# Autodesk Inventor assembly: AM14U3 Wide Frame Wheel mount
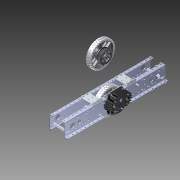
[picture p0: Inventor's stored thumbnail of the model, 180x180]
Saved by Autodesk Inventor 2014 (Build 180170000, 170)
## iProperties
Created: 2016-01-19
Part Number: AM14U3 Wide Frame Wheel mount
Document SubType Name: Assembly
Designer: choices
Author: choices
## Documents named in this file (12)
- F:\Robotics who knows idk\2016 Robot CAD Files\AndyMark Chassis things\AM14U3 Wide Frame Wheel mount.iam
- F:\Robotics who knows idk\2016 Robot CAD Files\AndyMark Chassis things\Churro 3375.ipt
- F:\Robotics who knows idk\2016 Robot CAD Files\AndyMark Chassis things\FHTS 0.25-20-0.75_FHTS 0.25-20-G-0.75-C.ipt
- F:\Robotics who knows idk\2016 Robot CAD Files\AndyMark Chassis things\10-32x0500_shcs_HX-SHCS 0.19-32x1.375x1-C.ipt
- F:\Robotics who knows idk\2016 Robot CAD Files\AndyMark Chassis things\10-32 Nylock Nut.ipt
- F:\Robotics who knows idk\2016 Robot CAD Files\AndyMark Chassis things\AM14U3 Outside Sheet Wide.ipt
- F:\Robotics who knows idk\2016 Robot CAD Files\AndyMark Chassis things\AM14U3 Inside Sheet Wide.ipt
- F:\Robotics who knows idk\2016 Robot CAD Files\AndyMark Chassis things\am-2954 AM14U2 2x3 Hole Bracket.ipt
- F:\Robotics who knows idk\2016 Robot CAD Files\AndyMark Chassis things\6 HiGrip with hub and double pulley.iam
- F:\Robotics who knows idk\2016 Robot CAD Files\AndyMark Chassis things\FR8ZZ Hex Bearing.ipt
- F:\Robotics who knows idk\2016 Robot CAD Files\AndyMark Chassis things\am-2598_107 2016 KOP Toughbox Mini.iam
- F:\Robotics who knows idk\2016 Robot CAD Files\AndyMark Chassis things\6 HiGrip with bearings, pulleys and spacers.iam
## Components (47 placed, 47 different names)
1. Churro 3375_80
2. Churro 3375_81
3. Churro 3375_82
4. Churro 3375_83
5. FHTS 0.25-20-0.75_FHTS 0.25-20-G-0.75-C_85
6. FHTS 0.25-20-0.75_FHTS 0.25-20-G-0.75-C_86
7. FHTS 0.25-20-0.75_FHTS 0.25-20-G-0.75-C_87
8. FHTS 0.25-20-0.75_FHTS 0.25-20-G-0.75-C_88
9. FHTS 0.25-20-0.75_FHTS 0.25-20-G-0.75-C_89
10. FHTS 0.25-20-0.75_FHTS 0.25-20-G-0.75-C_90
11. FHTS 0.25-20-0.75_FHTS 0.25-20-G-0.75-C_91
12. FHTS 0.25-20-0.75_FHTS 0.25-20-G-0.75-C_92
13. FHTS 0.25-20-0.75_FHTS 0.25-20-G-0.75-C_93
14. 10-32x0500_shcs_HX-SHCS 0.19-32x1.375x1-C_95
15. 10-32x0500_shcs_HX-SHCS 0.19-32x1.375x1-C_96
16. 10-32x0500_shcs_HX-SHCS 0.19-32x1.375x1-C_97
17. 10-32x0500_shcs_HX-SHCS 0.19-32x1.375x1-C_98
18. 10-32x0500_shcs_HX-SHCS 0.19-32x1.375x1-C_99
19. 10-32x0500_shcs_HX-SHCS 0.19-32x1.375x1-C_100
20. 10-32x0500_shcs_HX-SHCS 0.19-32x1.375x1-C_101
21. 10-32x0500_shcs_HX-SHCS 0.19-32x1.375x1-C_102
22. 10-32x0500_shcs_HX-SHCS 0.19-32x1.375x1-C_103
23. 10-32x0500_shcs_HX-SHCS 0.19-32x1.375x1-C_104
24. 10-32x0500_shcs_HX-SHCS 0.19-32x1.375x1-C_105
25. 10-32x0500_shcs_HX-SHCS 0.19-32x1.375x1-C_106
26. 10-32x0500_shcs_HX-SHCS 0.19-32x1.375x1-C_107
27. 10-32 Nylock Nut_113
28. 10-32 Nylock Nut_114
29. 10-32 Nylock Nut_115
30. 10-32 Nylock Nut_116
31. 10-32 Nylock Nut_117
32. 10-32 Nylock Nut_118
33. 10-32 Nylock Nut_119
34. 10-32 Nylock Nut_120
35. 10-32 Nylock Nut_121
36. 10-32 Nylock Nut_122
37. 10-32 Nylock Nut_123
38. 10-32 Nylock Nut_124
39. 10-32 Nylock Nut_125
40. AM14U3 Outside Sheet Wide_132 — Mate:6, Mate:10
41. AM14U3 Inside Sheet Wide_133 — Mate:3, Mate:4, Mate:5
42. am-2954 AM14U2 2x3 Hole Bracket_134
43. am-2954 AM14U2 2x3 Hole Bracket_135
44. 6 HiGrip with hub and double pulley:1 [sub-assembly] — Mate:7, Mate:8, Mate:9
45. am-2598_107 2016 KOP Toughbox Mini:1 [sub-assembly] — Mate:3, Mate:4, Mate:5, Mate:8, Mate:9
46. FR8ZZ Hex Bearing:1 — Mate:6, Mate:7, Mate:10
47. 6 HiGrip with bearings, pulleys and spacers:1 [sub-assembly]
## Relationships (8: Mate 8)
- Mate:3: AM14U3 Inside Sheet Wide_133 ↔ am-2598_107 2016 KOP Toughbox Mini:1
- Mate:4: AM14U3 Inside Sheet Wide_133 ↔ am-2598_107 2016 KOP Toughbox Mini:1
- Mate:5: AM14U3 Inside Sheet Wide_133 ↔ am-2598_107 2016 KOP Toughbox Mini:1
- Mate:6: AM14U3 Outside Sheet Wide_132 ↔ FR8ZZ Hex Bearing:1
- Mate:7: 6 HiGrip with hub and double pulley:1 ↔ FR8ZZ Hex Bearing:1
- Mate:8: 6 HiGrip with hub and double pulley:1 ↔ am-2598_107 2016 KOP Toughbox Mini:1
- Mate:9: 6 HiGrip with hub and double pulley:1 ↔ am-2598_107 2016 KOP Toughbox Mini:1
- Mate:10: AM14U3 Outside Sheet Wide_132 ↔ FR8ZZ Hex Bearing:1
